# Autodesk Inventor assembly: tank_separator_assembly
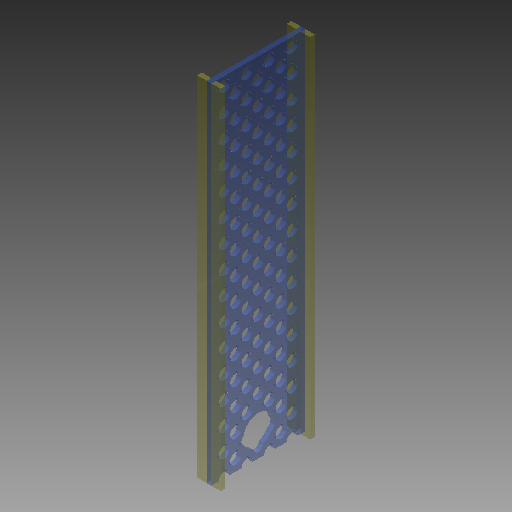
[picture p0: Inventor's stored thumbnail of the model, 512x512]
Saved by Autodesk Inventor 2018.1 (Build 221171000, 171)
## iProperties
Created: 2017-08-15
Part Number: tank_separator_assembly
Document SubType Name: Assembly
Designer: Tom
Mass: 206.463 g
Surface Area: 1086.78 cm^2
Volume: 147.474 cm^3
Density: 1.4 g/cm^3
Author: Tom
## Documents named in this file (4)
- \\Mac\Dropbox\2015-2016\Bachelorproef\Inventor\Etstank_v2\tank_separator_assembly.iam
- \\Mac\Dropbox\2015-2016\Bachelorproef\Inventor\Etstank_v2\tank_separator.ipt
- \\Mac\Dropbox\2015-2016\Bachelorproef\Inventor\Etstank_v2\tank_bracket_long.ipt
- \\Mac\Dropbox\2015-2016\Bachelorproef\Inventor\Etstank_v2\par.xls
## Components (5 placed, 2 different names)
1. tank_separator:1 — Mate:1, Mate:2, Mate:3, Mate:4, Flush:1, Flush:2, Flush:3, Flush:4, Flush:5, Flush:6, Flush:7, Flush:8
2. tank_bracket_long:1 — Mate:2, Flush:1, Flush:7
3. tank_bracket_long:2 — Mate:1, Flush:2, Flush:8
4. tank_bracket_long:3 — Mate:3, Flush:3, Flush:6
5. tank_bracket_long:4 — Mate:4, Flush:4, Flush:5
## Relationships (12: Flush 8, Mate 4)
- Mate:1: tank_separator:1 ↔ tank_bracket_long:2
- Mate:2: tank_separator:1 ↔ tank_bracket_long:1
- Mate:3: tank_separator:1 ↔ tank_bracket_long:3
- Mate:4: tank_separator:1 ↔ tank_bracket_long:4
- Flush:1: tank_separator:1 ↔ tank_bracket_long:1
- Flush:2: tank_separator:1 ↔ tank_bracket_long:2
- Flush:3: tank_separator:1 ↔ tank_bracket_long:3
- Flush:4: tank_separator:1 ↔ tank_bracket_long:4
- Flush:5: tank_separator:1 ↔ tank_bracket_long:4
- Flush:6: tank_separator:1 ↔ tank_bracket_long:3
- Flush:7: tank_separator:1 ↔ tank_bracket_long:1
- Flush:8: tank_separator:1 ↔ tank_bracket_long:2
## Named parameters: maxl = 400 mm, maxh = 400 mm, maxw = 350 mm, lcsd = 19.05 mm, lcdd = 100 mm, lcwd1 = 25 mm, lcwd2 = 34 mm, lcw = 20 mm, lch1 = 39 mm, lch2 = 40 mm, lcl = 150 mm, lcwd3 = 43 mm, dia1 = 6 mm, td = 18 mm, bhh = 6 mm, bhd = 10 mm, sw = 25 mm, sh = 31 mm, spacert = 2 mm, nutdist = 40 mm, platft = 20 mm, supt = 20 mm, pvct = 5 mm, tankw = 100 mm, tankh = 370 mm, tankl = 379 mm, dia2 = 20 mm, tankv = 1e+07 mm, actual_tankv = 1.4023e+07 mm, dia4 = 11 mm, dia3 = 8 mm, play = 9 mm, holeh = 26 mm, surroundh = 60 mm, slack = 0.5 mm, surroundt = 5 mm, play2 = 3 mm, extra_height = 100 mm, diaair = 32 mm, diaph = 32 mm, diawater = 25 mm, diacucl = 32 mm, diafloat = 50 mm, diahcl = 32 mm, diaoverflow = 25 mm, mindist = 80 mm, distfromedge = 10 mm, diasurroundhole = 42 mm, bracketw = 10 mm, bracketwbottom = 6 mm, sensorsupportl = 100 mm, diagrate = 12 mm, gratespacing = 12.02082 mm, bottomdist = 9.6355 mm, sidedist = 13.9375 mm, handlew = 50 mm, handlel = 120 mm, handlesupporth = 20 mm, nutholdert = 10 mm, nett = 1 mm, netholespacing = 2 mm, nethole = 16 mm, netside = 3.5 mm, nettop = 7 mm, diaetape = 32 mm
